# Autodesk Inventor assembly: V2
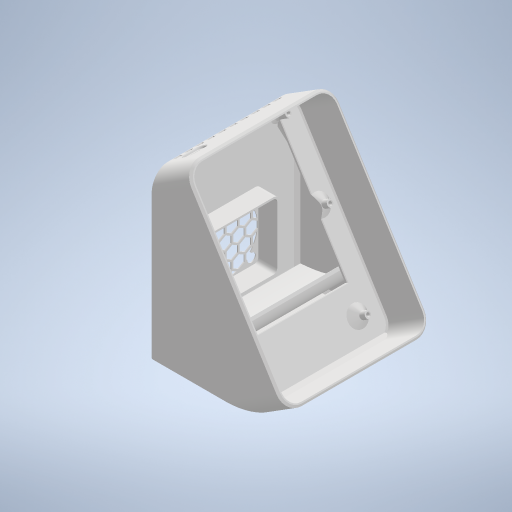
[picture p0: Inventor's stored thumbnail of the model, 512x512]
Saved by Autodesk Inventor 2023.1 (Build 271208000, 208)
## iProperties
Created: 2022-09-10
Part Number: V2
Document SubType Name: Assembly
Designer: Rama
Author: Rama
## Documents named in this file (3)
- C:\Users\Rama\Desktop\GitHub\Voron-2-Mods\Misc\ISDT C4 EVO\CAD\Housing.iam
- C:\Users\Rama\Desktop\GitHub\Voron-2-Mods\Misc\ISDT C4 EVO\CAD\SRC\FanCover.ipt
- C:\Users\Rama\Desktop\GitHub\Voron-2-Mods\Misc\ISDT C4 EVO\CAD\SRC\Housing.ipt
## Components (2 placed, 2 different names)
1. FanCover:1 — Fluchtend:1, Passend:1, Passend:2
2. Housing:1 — Fluchtend:1, Passend:1, Passend:2, Passend:3, Passend:4, Passend:5
## Relationships (6: Mate 5, Flush 1)
- Fluchtend:1 [Flush]: FanCover:1 ↔ Housing:1
- Passend:1 [Mate]: FanCover:1 ↔ Housing:1
- Passend:2 [Mate]: FanCover:1 ↔ Housing:1
- Passend:3 [Mate]: Housing:1
- Passend:4 [Mate]: Housing:1
- Passend:5 [Mate]: Housing:1
